# Autodesk Inventor assembly: CoreXY Idler 4040 Assembly Left V2
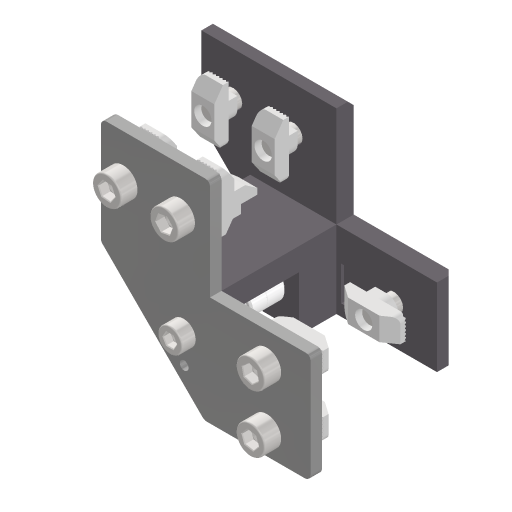
[picture p0: Inventor's stored thumbnail of the model, 512x512]
Saved by Autodesk Inventor 2023.2 (Build 272271000, 271)
## iProperties
Created: 2023-11-27
Part Number: CoreXY Idler 4040 Assembly Left V2
Document SubType Name: Assembly
Designer: Nils Bade
Author: Nils Bade
## Documents named in this file (13)
- C:\Users\nilsb\Documents\Inventor\Projektarbeit-Bade\RatRig_Bade\CoreXY Idler 4040 Assembly Left V2.iam
- C:\Users\nilsb\Documents\Inventor\Projektarbeit-Bade\RatRig_modified\Idler Plate for 4040.ipt
- C:\Users\nilsb\Documents\Inventor\Projektarbeit-Bade\RatRig_Standards\Hex Locking Nut - M5 v2.ipt
- C:\Users\nilsb\Documents\Inventor\Projektarbeit-Bade\RatRig_modified\T-NUT - DropIn 4040 SERIES - M6.ipt
- C:\Users\nilsb\Documents\Inventor\Projektarbeit-Bade\Schrauben\Cap Head Screw M6x16.ipt
- C:\Users\nilsb\Documents\Inventor\Projektarbeit-Bade\Schrauben\Cap Head Screw M6x12 v2.ipt
- C:\Users\nilsb\Documents\Inventor\Projektarbeit-Bade\Schrauben\Countersink Screw M6x14 v2.ipt
- C:\Users\nilsb\Documents\Inventor\Projektarbeit-Bade\RatRig_Standards\Mini Precision Shim - 8x5x1mm v2.ipt
- C:\Users\nilsb\Documents\Inventor\Projektarbeit-Bade\RatRig_Standards\Ball Bearing - F695ZZ v1.ipt
- C:\Users\nilsb\Documents\Inventor\Projektarbeit-Bade\RatRig_Standards\Ball Bearing - 695ZZ v1.ipt
- C:\Users\nilsb\Documents\Inventor\Projektarbeit-Bade\RatRig_Standards\Aluminium Spacer - 6mm v2.ipt
- C:\Users\nilsb\Documents\Inventor\Projektarbeit-Bade\RatRig_modified\xy Idler Left for 4040 V2.ipt
- C:\Users\nilsb\Documents\Inventor\Projektarbeit-Bade\Schrauben\Cap Head Screw M5x50.ipt
## Components (28 placed, 12 different names)
1. xy Idler Left for 4040 2:1 — Passend:61, Passend:62
2. Idler Plate for 4040:1 — Passend:11, Passend:12, Passend:13, Passend:14, Winkel:1, Winkel:2, Winkel:3, Winkel:4, Passend:16, Passend:19, Passend:20, Passend:21, Passend:28, Passend:29, Passend:30, Passend:31, Passend:32, Passend:33, Passend:34, Passend:35, Passend:45
3. Cap Head Screw M5x50:1
4. Hex Locking Nut - M5 v2:1
5. T-NUT - DROP IN TYPE FOR 40 SERIES - M6:1 — Passend:11, Winkel:4, Passend:16
6. T-NUT - DROP IN TYPE FOR 40 SERIES - M6:2 — Passend:12, Winkel:3, Passend:19
7. T-NUT - DROP IN TYPE FOR 40 SERIES - M6:3 — Passend:13, Winkel:2, Passend:20
8. T-NUT - DROP IN TYPE FOR 40 SERIES - M6:4 — Passend:14, Winkel:1, Passend:21
9. T-NUT - DROP IN TYPE FOR 40 SERIES - M6:5
10. T-NUT - DROP IN TYPE FOR 40 SERIES - M6:6 — Passend:10
11. T-NUT - DROP IN TYPE FOR 40 SERIES - M6:7
12. T-NUT - DROP IN TYPE FOR 40 SERIES - M6:9 — Passend:7
13. Cap Head Screw M6x16:1 — Passend:61, Passend:62
14. Cap Head Screw M6x12 v2:1 — Passend:29, Passend:33
15. Cap Head Screw M6x12 v2:2 — Passend:28, Passend:32
16. Cap Head Screw M6x12 v2:3 — Passend:31, Passend:35
17. Cap Head Screw M6x12 v2:4 — Passend:30, Passend:34
18. Countersink Screw M6x14 v2:1
19. Countersink Screw M6x14 v2:2 — Passend:10
20. Countersink Screw M6x14 v2:4 — Passend:7
21. Mini Precision Shim - 8x5x1mm v2:1 — Passend:45, Passend:54
22. Mini Precision Shim - 8x5x1mm v2:2 — Passend:53, Passend:58
23. Mini Precision Shim - 8x5x1mm v2:3 — Passend:60
24. Ball Bearing - F695ZZ v1:1 — Passend:51, Passend:53
25. Ball Bearing - F695ZZ v1:2 — Passend:49, Passend:54
26. Ball Bearing - 695ZZ v1:1 — Passend:49, Passend:51
27. Aluminium Spacer - 6mm v2:1 — Passend:59, Passend:60
28. Aluminium Spacer - 6mm v2:2 — Passend:58, Passend:59
## Relationships (64: Mate 53, Angle 9, Flush 2)
- [Flush]: xy Idler Left for 4040 2:1 ↔ Idler Plate for 4040:1
- [Flush]: xy Idler Left for 4040 2:1 ↔ Idler Plate for 4040:1
- [Mate]: xy Idler Left for 4040 2:1 ↔ Idler Plate for 4040:1
- [Mate]: Idler Plate for 4040:1 ↔ Cap Head Screw M5x50:1
- [Mate]: Idler Plate for 4040:1 ↔ Cap Head Screw M5x50:1
- [Mate]: Cap Head Screw M5x50:1 ↔ Hex Locking Nut - M5 v2:1
- [Mate]: xy Idler Left for 4040 2:1 ↔ Hex Locking Nut - M5 v2:1
- Passend:7 [Mate]: T-NUT - DROP IN TYPE FOR 40 SERIES - M6:9 ↔ Countersink Screw M6x14 v2:4
- [Mate]: xy Idler Left for 4040 2:1 ↔ T-NUT - DROP IN TYPE FOR 40 SERIES - M6:7
- Passend:10 [Mate]: T-NUT - DROP IN TYPE FOR 40 SERIES - M6:6 ↔ Countersink Screw M6x14 v2:2
- Passend:11 [Mate]: Idler Plate for 4040:1 ↔ T-NUT - DROP IN TYPE FOR 40 SERIES - M6:1
- Passend:12 [Mate]: Idler Plate for 4040:1 ↔ T-NUT - DROP IN TYPE FOR 40 SERIES - M6:2
- Passend:13 [Mate]: Idler Plate for 4040:1 ↔ T-NUT - DROP IN TYPE FOR 40 SERIES - M6:3
- Passend:14 [Mate]: Idler Plate for 4040:1 ↔ T-NUT - DROP IN TYPE FOR 40 SERIES - M6:4
- Winkel:1 [Angle] (0 deg): Idler Plate for 4040:1 ↔ T-NUT - DROP IN TYPE FOR 40 SERIES - M6:4
- Winkel:2 [Angle] (0 deg): Idler Plate for 4040:1 ↔ T-NUT - DROP IN TYPE FOR 40 SERIES - M6:3
- Winkel:3 [Angle] (0 deg): Idler Plate for 4040:1 ↔ T-NUT - DROP IN TYPE FOR 40 SERIES - M6:2
- Winkel:4 [Angle] (0 deg): Idler Plate for 4040:1 ↔ T-NUT - DROP IN TYPE FOR 40 SERIES - M6:1
- [Angle] (0 deg): xy Idler Left for 4040 2:1 ↔ T-NUT - DROP IN TYPE FOR 40 SERIES - M6:5
- Passend:16 [Mate] (5.5 mm): Idler Plate for 4040:1 ↔ T-NUT - DROP IN TYPE FOR 40 SERIES - M6:1
- [Mate]: xy Idler Left for 4040 2:1 ↔ T-NUT - DROP IN TYPE FOR 40 SERIES - M6:5
- [Mate] (5.5 mm): xy Idler Left for 4040 2:1 ↔ T-NUT - DROP IN TYPE FOR 40 SERIES - M6:5
- Passend:19 [Mate] (5.5 mm): Idler Plate for 4040:1 ↔ T-NUT - DROP IN TYPE FOR 40 SERIES - M6:2
- Passend:20 [Mate] (5.5 mm): Idler Plate for 4040:1 ↔ T-NUT - DROP IN TYPE FOR 40 SERIES - M6:3
- Passend:21 [Mate] (5.5 mm): Idler Plate for 4040:1 ↔ T-NUT - DROP IN TYPE FOR 40 SERIES - M6:4
- [Angle] (0 deg): xy Idler Left for 4040 2:1 ↔ T-NUT - DROP IN TYPE FOR 40 SERIES - M6:9
- [Angle] (0 deg): xy Idler Left for 4040 2:1 ↔ T-NUT - DROP IN TYPE FOR 40 SERIES - M6:7
- [Angle] (0 deg): xy Idler Left for 4040 2:1 ↔ T-NUT - DROP IN TYPE FOR 40 SERIES - M6:6
- [Mate] (5.5 mm): xy Idler Left for 4040 2:1 ↔ T-NUT - DROP IN TYPE FOR 40 SERIES - M6:6
- [Mate] (5.5 mm): xy Idler Left for 4040 2:1 ↔ T-NUT - DROP IN TYPE FOR 40 SERIES - M6:7
- [Mate] (5.5 mm): xy Idler Left for 4040 2:1 ↔ T-NUT - DROP IN TYPE FOR 40 SERIES - M6:9
- Passend:28 [Mate]: Idler Plate for 4040:1 ↔ Cap Head Screw M6x12 v2:2
- Passend:29 [Mate]: Idler Plate for 4040:1 ↔ Cap Head Screw M6x12 v2:1
- Passend:30 [Mate]: Idler Plate for 4040:1 ↔ Cap Head Screw M6x12 v2:4
- Passend:31 [Mate]: Idler Plate for 4040:1 ↔ Cap Head Screw M6x12 v2:3
- Passend:32 [Mate]: Idler Plate for 4040:1 ↔ Cap Head Screw M6x12 v2:2
- Passend:33 [Mate]: Idler Plate for 4040:1 ↔ Cap Head Screw M6x12 v2:1
- Passend:34 [Mate]: Idler Plate for 4040:1 ↔ Cap Head Screw M6x12 v2:4
- Passend:35 [Mate]: Idler Plate for 4040:1 ↔ Cap Head Screw M6x12 v2:3
- [Mate]: xy Idler Left for 4040 2:1 ↔ Countersink Screw M6x14 v2:4
- [Mate]: xy Idler Left for 4040 2:1 ↔ Countersink Screw M6x14 v2:1
- [Mate]: xy Idler Left for 4040 2:1 ↔ Countersink Screw M6x14 v2:2
- [Mate]: xy Idler Left for 4040 2:1 ↔ Countersink Screw M6x14 v2:4
- [Mate]: xy Idler Left for 4040 2:1 ↔ Countersink Screw M6x14 v2:1
- [Mate]: xy Idler Left for 4040 2:1 ↔ Countersink Screw M6x14 v2:2
- [Mate]: Cap Head Screw M5x50:1 ↔ Mini Precision Shim - 8x5x1mm v2:1
- Passend:45 [Mate]: Idler Plate for 4040:1 ↔ Mini Precision Shim - 8x5x1mm v2:1
- [Mate]: Cap Head Screw M5x50:1 ↔ Ball Bearing - F695ZZ v1:2
- [Mate]: Cap Head Screw M5x50:1 ↔ Ball Bearing - 695ZZ v1:1
- Passend:49 [Mate]: Ball Bearing - F695ZZ v1:2 ↔ Ball Bearing - 695ZZ v1:1
- [Mate]: Cap Head Screw M5x50:1 ↔ Ball Bearing - F695ZZ v1:1
- Passend:51 [Mate]: Ball Bearing - F695ZZ v1:1 ↔ Ball Bearing - 695ZZ v1:1
- [Mate]: Cap Head Screw M5x50:1 ↔ Mini Precision Shim - 8x5x1mm v2:2
- Passend:53 [Mate]: Mini Precision Shim - 8x5x1mm v2:2 ↔ Ball Bearing - F695ZZ v1:1
- Passend:54 [Mate]: Mini Precision Shim - 8x5x1mm v2:1 ↔ Ball Bearing - F695ZZ v1:2
- [Mate]: Cap Head Screw M5x50:1 ↔ Aluminium Spacer - 6mm v2:2
- [Mate]: Cap Head Screw M5x50:1 ↔ Aluminium Spacer - 6mm v2:1
- [Mate]: Cap Head Screw M5x50:1 ↔ Mini Precision Shim - 8x5x1mm v2:3
- Passend:58 [Mate]: Mini Precision Shim - 8x5x1mm v2:2 ↔ Aluminium Spacer - 6mm v2:2
- Passend:59 [Mate]: Aluminium Spacer - 6mm v2:1 ↔ Aluminium Spacer - 6mm v2:2
- Passend:60 [Mate]: Mini Precision Shim - 8x5x1mm v2:3 ↔ Aluminium Spacer - 6mm v2:1
- [Angle] (0 deg): xy Idler Left for 4040 2:1 ↔ Hex Locking Nut - M5 v2:1
- Passend:61 [Mate]: xy Idler Left for 4040 2:1 ↔ Cap Head Screw M6x16:1
- Passend:62 [Mate]: xy Idler Left for 4040 2:1 ↔ Cap Head Screw M6x16:1
